# Autodesk Inventor assembly: SchiffsschraubeBaugruppe.ipt
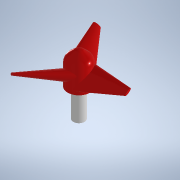
[picture p0: Inventor's stored thumbnail of the model, 180x180]
Saved by Autodesk Inventor 2021 (Build 250183000, 183)
## iProperties
Created: 2021-01-29
Part Number: SchiffsschraubeBaugruppe.ipt
Document SubType Name: Assembly
Designer: LETPJG
Author: LETPJG
## Documents named in this file (3)
- C:\Users\LETPJG\Documents\Vault\Gruppen\Gruppe 2\Entwurf\Amphibienfahrzeug\SchiffsschraubeBaugruppe.ipt.iam
- C:\Users\LETPJG\Documents\Vault\Gruppen\Gruppe 2\Entwurf\Amphibienfahrzeug\BauteilWelle1.ipt
- C:\Users\LETPJG\Documents\Vault\Gruppen\Gruppe 2\Entwurf\Amphibienfahrzeug\Schiffsschraube.ipt
## Components (2 placed, 2 different names)
1. BauteilWelle1:1 — Einfügen:2
2. Schiffsschraube:1 — Einfügen:2
## Relationships (1: Insert 1)
- Einfügen:2 [Insert]: BauteilWelle1:1 ↔ Schiffsschraube:1
